# Autodesk Inventor assembly: thumper-bumper-assm-v3
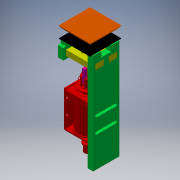
[picture p0: Inventor's stored thumbnail of the model, 180x180]
Saved by Autodesk Inventor 2017 (Build 210142000, 142)
## iProperties
Created: 2017-02-23
Part Number: thumper-bumper-assm-v3
Document SubType Name: Assembly
Designer: John
Author: John
## Documents named in this file (9)
- C:\Users\John\Dropbox\ECE115\pinball-project\thumper-bumper-assm-v3.iam
- C:\Users\John\Dropbox\ECE115\pinball-project\thumper-base-v3.ipt
- C:\Users\John\Dropbox\ECE115\pinball-project\thumper-bumper-sidewall2-v3.ipt
- C:\Users\John\Dropbox\ECE115\pinball-project\thumper-bumper-sidewall-v3.ipt
- C:\Users\John\Dropbox\ECE115\module-2\Solenoid 1240S\Solenoid.iam
- C:\Users\John\Dropbox\ECE115\pinball-project\thumper-bumper-top-v3.ipt
- C:\Users\John\Dropbox\ECE115\pinball-project\thumper-bumper-trigger-v2.ipt
- C:\Users\John\Dropbox\ECE115\pinball-project\thumper-bumper-plunger.ipt
- C:\Users\John\Dropbox\ECE115\pinball-project\thumper-bumper-plunger-interface.ipt
## Components (9 placed, 8 different names)
1. thumper-base-v3:1 — Flush:1, Mate:1, Flush:3, Mate:6, Angle:2, Mate:11, Angle:4, Insert:3, Angle:5, Mate:21
2. thumper-bumper-sidewall2-v3:1 — Flush:1, Mate:1, Mate:18, Mate:19, Flush:5, Mate:21
3. thumper-bumper-sidewall-v3:1 — Flush:3, Mate:6, Insert:2
4. Solenoid:1 [sub-assembly] — Insert:2, Angle:2, Mate:20, Insert:4, Angle:6
5. thumper-bumper-top-v3:1 — Mate:18, Mate:19, Flush:5, Cylindrical:1
6. thumper-bumper-trigger-v2:1 — Mate:11, Angle:4, Insert:3
7. thumper-bumper-plunger:1 — Mate:20, Cylindrical:1, Angle:5, Rigid:1
8. thumper-bumper-plunger-interface:1 — Insert:4, Angle:6
9. thumper-bumper-plunger-interface:2 — Rigid:1
## Relationships (19: Mate 7, Angle 4, Flush 3, Insert 3, CylindricalJoint 1, WeldJoint 1)
- Flush:1: thumper-base-v3:1 ↔ thumper-bumper-sidewall2-v3:1
- Mate:1: thumper-base-v3:1 ↔ thumper-bumper-sidewall2-v3:1
- Flush:3: thumper-base-v3:1 ↔ thumper-bumper-sidewall-v3:1
- Mate:6: thumper-base-v3:1 ↔ thumper-bumper-sidewall-v3:1
- Insert:2: thumper-bumper-sidewall-v3:1 ↔ Solenoid:1
- Angle:2 (180 deg): thumper-base-v3:1 ↔ Solenoid:1
- Mate:11: thumper-base-v3:1 ↔ thumper-bumper-trigger-v2:1
- Mate:18: thumper-bumper-sidewall2-v3:1 ↔ thumper-bumper-top-v3:1
- Mate:19: thumper-bumper-sidewall2-v3:1 ↔ thumper-bumper-top-v3:1
- Flush:5: thumper-bumper-sidewall2-v3:1 ↔ thumper-bumper-top-v3:1
- Angle:4 (180 deg): thumper-base-v3:1 ↔ thumper-bumper-trigger-v2:1
- Insert:3 (0.5 mm): thumper-base-v3:1 ↔ thumper-bumper-trigger-v2:1
- Mate:20 (1 mm): Solenoid:1 ↔ thumper-bumper-plunger:1
- Cylindrical:1: thumper-bumper-top-v3:1 ↔ thumper-bumper-plunger:1
- Angle:5 (0 deg): thumper-base-v3:1 ↔ thumper-bumper-plunger:1
- Insert:4: Solenoid:1 ↔ thumper-bumper-plunger-interface:1
- Angle:6 (180 deg): Solenoid:1 ↔ thumper-bumper-plunger-interface:1
- Rigid:1 [WeldJoint]: thumper-bumper-plunger:1 ↔ thumper-bumper-plunger-interface:2
- Mate:21: thumper-base-v3:1 ↔ thumper-bumper-sidewall2-v3:1
